# Autodesk Inventor assembly: left_gripper_whole
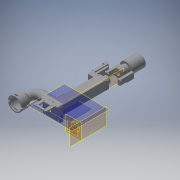
[picture p0: Inventor's stored thumbnail of the model, 180x180]
Saved by Autodesk Inventor 2016 (Build 200138000, 138)
## iProperties
Created: 2016-06-09
Part Number: left_gripper_whole
Material: 一般
Document SubType Name: Assembly
Designer: Shun Hasegawa
Author: Shun Hasegawa
## Documents named in this file (3)
- C:\Shun\AmazonPickingChallenge\test3\left\left_gripper_whole.iam
- C:\Shun\AmazonPickingChallenge\test3\left\left_gripper_base.iam
- C:\Shun\AmazonPickingChallenge\test3\left\left_gripper_cup_with_base.iam
## Components (2 placed, 2 different names)
1. left_gripper_base:1 [sub-assembly] — メイト:1, 角度:1
2. left_gripper_cup_with_base:1 [sub-assembly] — メイト:1, メイト:2, 角度:1
## Relationships (3: Mate 2, Angle 1)
- メイト:1 [Mate]: left_gripper_base:1 ↔ left_gripper_cup_with_base:1
- メイト:2 [Mate]: left_gripper_cup_with_base:1
- 角度:1 [Angle] (0 deg): left_gripper_base:1 ↔ left_gripper_cup_with_base:1
